# Autodesk Inventor assembly: ロボット回転
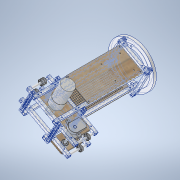
[picture p0: Inventor's stored thumbnail of the model, 180x180]
Saved by Autodesk Inventor 2020.3 (Build 243373000, 373)
## iProperties
Created: 2020-07-04
Part Number: ロボット回転
Document SubType Name: Assembly
Designer: totot
Mass: 887.957 g
Surface Area: 3001.88 cm^2
Volume: 382.741 cm^3
Density: 2.32 g/cm^3
Author: totot
## Documents named in this file (20)
- D:\mysvn\ロボコン\キャチロボ\キャチロボ設計図\ロボット\ハンド\ロボット回転.iam
- D:\mysvn\ロボコン\キャチロボ\キャチロボ設計図\ロボット\共有パーツ\turntable1.ipt
- D:\mysvn\ロボコン\キャチロボ\キャチロボ設計図\ロボット\共有パーツ\turntable2.ipt
- D:\mysvn\ロボコン\キャチロボ\キャチロボ設計図\ロボット\ハンド\ロボット回転9ｘ9_1.ipt
- D:\mysvn\ロボコン\キャチロボ\キャチロボ設計図\ロボット\ハンド\ロボット回転9x9_2.ipt
- D:\mysvn\ロボコン\キャチロボ\キャチロボ設計図\ロボット\ハンド\ロボット回転9x9_3.ipt
- D:\mysvn\ロボコン\キャチロボ\キャチロボ設計図\ロボット\ハンド\ロボット回転t5.5.ipt
- D:\mysvn\ロボコン\キャチロボ\キャチロボ設計図\ロボット\共有パーツ\RS_540.ipt
- D:\mysvn\ロボコン\キャチロボ\キャチロボ設計図\ロボット\共有パーツ\PS1-20_On.ipt
- D:\mysvn\ロボコン\キャチロボ\キャチロボ設計図\ロボット\ハンド\ロボット回転_ベアリングシャフト縦.ipt
- D:\mysvn\ロボコン\キャチロボ\キャチロボ設計図\ロボット\ハンド\ロボット回転_ベアリングシャフト横.ipt
- D:\mysvn\ロボコン\キャチロボ\キャチロボ設計図\ロボット\ハンド\ロボット回転9x9_4.ipt
- D:\mysvn\ロボコン\キャチロボ\キャチロボ設計図\ロボット\ハンド\ハンド_ベアリング_4-8.ipt
- D:\mysvn\ロボコン\キャチロボ\キャチロボ設計図\ロボット\共有パーツ\ベアリング_6-17.ipt
- D:\mysvn\ロボコン\キャチロボ\キャチロボ設計図\ロボット\共有パーツ\ロボット回転_回路ボード1.ipt
- D:\mysvn\ロボコン\キャチロボ\キャチロボ設計図\ロボット\共有パーツ\ロボット回転_回路ボード1_CPY.ipt
- D:\mysvn\ロボコン\キャチロボ\キャチロボ設計図\ロボット\共有パーツ\AMT102-Vwide.ipt
- D:\mysvn\ロボコン\キャチロボ\キャチロボ設計図\ロボット\上下直動\ロボット回転t5.5_2.ipt
- D:\mysvn\ロボコン\キャチロボ\キャチロボ設計図\ロボット\上下直動\ロボット回転_エンコーダシャフト.ipt
- D:\mysvn\ロボコン\キャチロボ\キャチロボ設計図\ロボット\共有パーツ\F606ZZ\F606ZZ.iam
## Components (44 placed, 19 different names)
1. turntable1:1 — 正接:1, フラッシュ:1
2. turntable2:1 — 正接:1, フラッシュ:1, 挿入:1, 挿入:2, 挿入:3, 挿入:4
3. ロボット回転9ｘ9_1:1 — 挿入:1, 挿入:2, 挿入:5, 挿入:7, 挿入:17
4. ロボット回転9ｘ9_1:2 — 挿入:3, 挿入:4, 挿入:6, 挿入:8, 挿入:20, 挿入:66
5. ロボット回転9ｘ9_1:3 — 挿入:7, 挿入:8
6. ロボット回転9ｘ9_1:4 — 挿入:5, 挿入:6, 挿入:18, 挿入:19
7. ロボット回転_ベアリングシャフト縦:1 — 正接:26, 正接:27
8. ロボット回転9x9_2:1 — 挿入:17, 挿入:18, 挿入:24, 角度:1, 挿入:48, 挿入:51, 挿入:60, 挿入:69, 挿入:70, 挿入:78
9. ロボット回転9x9_2:2 — 挿入:19, 挿入:20, 挿入:23, 挿入:49, 挿入:50, 挿入:54
10. ロボット回転9x9_3:1 — フラッシュ:6, 正接:6, 正接:7, フラッシュ:7, 挿入:48, 挿入:49, 挿入:55, 挿入:61
11. ロボット回転t5.5:1 — 挿入:23, 挿入:24, 挿入:25, 挿入:26, 挿入:52, 挿入:53, 挿入:71, 挿入:72
12. RS_540:1 — 挿入:25, 挿入:26, 正接:2, フラッシュ:2
13. PS1-20_On:1 — 正接:2, フラッシュ:2, メイト:12, フラッシュ:16
14. ロボット回転9x9_2:3 — 挿入:44, 挿入:46, 挿入:57, 挿入:66, 挿入:75
15. ロボット回転9x9_2:4 — 角度:1, 挿入:45, 挿入:47, 挿入:59, 挿入:67, 挿入:68, 挿入:77
16. ロボット回転9x9_3:2 — 挿入:46, 挿入:47, 正接:5, フラッシュ:5, 挿入:56, 挿入:58, 挿入:73
17. ロボット回転9x9_3:3 — 挿入:50, 挿入:51, メイト:14, 挿入:76
18. ロボット回転9x9_3:4 — 挿入:44, 挿入:45, 挿入:74
19. ロボット回転_ベアリングシャフト縦:2 — フラッシュ:6, 正接:6, 正接:23
20. ロボット回転_ベアリングシャフト縦:3 — 正接:5, フラッシュ:5, 正接:22
21. ロボット回転_ベアリングシャフト縦:4 — 正接:7, フラッシュ:7, 正接:24, 正接:28
22. ロボット回転_ベアリングシャフト横:1 — 挿入:52, 正接:21
23. ロボット回転_ベアリングシャフト横:2 — 挿入:53, 正接:20
24. ロボット回転9x9_4:1 — 挿入:54, 挿入:55, 挿入:56, 挿入:57
25. ロボット回転9x9_4:2 — 挿入:58, 挿入:59, 挿入:60, 挿入:61
26. ハンド_ベアリング_4-8:1 — メイト:10, 挿入:64
27. ハンド_ベアリング_4-8:2 — メイト:10, フラッシュ:8, 挿入:64, 正接:20, メイト:12
28. ハンド_ベアリング_4-8:3 — メイト:11, フラッシュ:8, 挿入:65
29. ハンド_ベアリング_4-8:4 — メイト:11, 挿入:65, 正接:21
30. ベアリング_6-17:1 — 正接:22, フラッシュ:12, フラッシュ:15
31. ベアリング_6-17:2 — フラッシュ:9, メイト:13, 正接:27, フラッシュ:15
32. ベアリング_6-17:3 — フラッシュ:14, 正接:24, メイト:14
33. ベアリング_6-17:5 — フラッシュ:14, 正接:26, メイト:13
34. ベアリング_6-17:6 — 正接:23, フラッシュ:12
35. ベアリング_6-17:7 — フラッシュ:9, 正接:28
36. ロボット回転_回路ボード1:1 — 挿入:67, 挿入:68
37. ロボット回転_回路ボード1_CPY:1 — 挿入:69, 挿入:70
38. AMT102-Vwide:1 — 挿入:71, 挿入:72, フラッシュ:17
39. PS1-20_On:2 — フラッシュ:16, 正接:30
40. ロボット回転t5.5_2:1 — 挿入:73, 挿入:74, 正接:31, メイト:15
41. ロボット回転_エンコーダシャフト:1 — フラッシュ:17, 正接:30, 正接:32
42. F606ZZ:1 [sub-assembly] — 正接:31, メイト:15, 正接:32
43. ロボット回転9x9_4:3 — 挿入:75, 挿入:76
44. ロボット回転9x9_4:4 — 挿入:77, 挿入:78
## Relationships (86: Insert 49, Tangent 17, Flush 13, Mate 6, Angle 1)
- 正接:1 [Tangent]: turntable1:1 ↔ turntable2:1
- フラッシュ:1 [Flush]: turntable1:1 ↔ turntable2:1
- 挿入:1 [Insert]: turntable2:1 ↔ ロボット回転9ｘ9_1:1
- 挿入:2 [Insert]: turntable2:1 ↔ ロボット回転9ｘ9_1:1
- 挿入:3 [Insert]: turntable2:1 ↔ ロボット回転9ｘ9_1:2
- 挿入:4 [Insert]: turntable2:1 ↔ ロボット回転9ｘ9_1:2
- 挿入:5 [Insert]: ロボット回転9ｘ9_1:1 ↔ ロボット回転9ｘ9_1:4
- 挿入:6 [Insert]: ロボット回転9ｘ9_1:2 ↔ ロボット回転9ｘ9_1:4
- 挿入:7 [Insert]: ロボット回転9ｘ9_1:1 ↔ ロボット回転9ｘ9_1:3
- 挿入:8 [Insert]: ロボット回転9ｘ9_1:2 ↔ ロボット回転9ｘ9_1:3
- 挿入:17 [Insert]: ロボット回転9ｘ9_1:1 ↔ ロボット回転9x9_2:1
- 挿入:18 [Insert]: ロボット回転9ｘ9_1:4 ↔ ロボット回転9x9_2:1
- 挿入:19 [Insert]: ロボット回転9ｘ9_1:4 ↔ ロボット回転9x9_2:2
- 挿入:20 [Insert]: ロボット回転9ｘ9_1:2 ↔ ロボット回転9x9_2:2
- 挿入:23 [Insert]: ロボット回転9x9_2:2 ↔ ロボット回転t5.5:1
- 挿入:24 [Insert]: ロボット回転9x9_2:1 ↔ ロボット回転t5.5:1
- 挿入:25 [Insert]: ロボット回転t5.5:1 ↔ RS_540:1
- 挿入:26 [Insert]: ロボット回転t5.5:1 ↔ RS_540:1
- 正接:2 [Tangent]: RS_540:1 ↔ PS1-20_On:1
- フラッシュ:2 [Flush] (-7 mm): RS_540:1 ↔ PS1-20_On:1
- 角度:1 [Angle] (-180 deg): ロボット回転9x9_2:1 ↔ ロボット回転9x9_2:4
- [Flush]: ロボット回転_ベアリングシャフト縦:1 ↔ ロボット回転9x9_3:4
- [Tangent]: ロボット回転_ベアリングシャフト縦:1 ↔ ロボット回転9x9_3:4
- 挿入:44 [Insert]: ロボット回転9x9_2:3 ↔ ロボット回転9x9_3:4
- 挿入:45 [Insert]: ロボット回転9x9_2:4 ↔ ロボット回転9x9_3:4
- 挿入:46 [Insert]: ロボット回転9x9_2:3 ↔ ロボット回転9x9_3:2
- 挿入:47 [Insert]: ロボット回転9x9_2:4 ↔ ロボット回転9x9_3:2
- 正接:5 [Tangent]: ロボット回転9x9_3:2 ↔ ロボット回転_ベアリングシャフト縦:3
- フラッシュ:5 [Flush]: ロボット回転9x9_3:2 ↔ ロボット回転_ベアリングシャフト縦:3
- フラッシュ:6 [Flush]: ロボット回転9x9_3:1 ↔ ロボット回転_ベアリングシャフト縦:2
- 正接:6 [Tangent]: ロボット回転9x9_3:1 ↔ ロボット回転_ベアリングシャフト縦:2
- 正接:7 [Tangent]: ロボット回転9x9_3:1 ↔ ロボット回転_ベアリングシャフト縦:4
- フラッシュ:7 [Flush]: ロボット回転9x9_3:1 ↔ ロボット回転_ベアリングシャフト縦:4
- 挿入:48 [Insert]: ロボット回転9x9_2:1 ↔ ロボット回転9x9_3:1
- 挿入:49 [Insert]: ロボット回転9x9_2:2 ↔ ロボット回転9x9_3:1
- 挿入:50 [Insert]: ロボット回転9x9_2:2 ↔ ロボット回転9x9_3:3
- 挿入:51 [Insert]: ロボット回転9x9_2:1 ↔ ロボット回転9x9_3:3
- 挿入:52 [Insert]: ロボット回転t5.5:1 ↔ ロボット回転_ベアリングシャフト横:1
- 挿入:53 [Insert]: ロボット回転t5.5:1 ↔ ロボット回転_ベアリングシャフト横:2
- 挿入:54 [Insert]: ロボット回転9x9_2:2 ↔ ロボット回転9x9_4:1
- 挿入:55 [Insert]: ロボット回転9x9_3:1 ↔ ロボット回転9x9_4:1
- 挿入:56 [Insert]: ロボット回転9x9_3:2 ↔ ロボット回転9x9_4:1
- 挿入:57 [Insert]: ロボット回転9x9_2:3 ↔ ロボット回転9x9_4:1
- 挿入:58 [Insert]: ロボット回転9x9_3:2 ↔ ロボット回転9x9_4:2
- 挿入:59 [Insert]: ロボット回転9x9_2:4 ↔ ロボット回転9x9_4:2
- 挿入:60 [Insert]: ロボット回転9x9_2:1 ↔ ロボット回転9x9_4:2
- 挿入:61 [Insert]: ロボット回転9x9_3:1 ↔ ロボット回転9x9_4:2
- メイト:10 [Mate]: ハンド_ベアリング_4-8:1 ↔ ハンド_ベアリング_4-8:2
- メイト:11 [Mate]: ハンド_ベアリング_4-8:3 ↔ ハンド_ベアリング_4-8:4
- フラッシュ:8 [Flush]: ハンド_ベアリング_4-8:2 ↔ ハンド_ベアリング_4-8:3
- 挿入:64 [Insert]: ハンド_ベアリング_4-8:1 ↔ ハンド_ベアリング_4-8:2
- 挿入:65 [Insert]: ハンド_ベアリング_4-8:3 ↔ ハンド_ベアリング_4-8:4
- 正接:20 [Tangent]: ロボット回転_ベアリングシャフト横:2 ↔ ハンド_ベアリング_4-8:2
- メイト:12 [Mate]: PS1-20_On:1 ↔ ハンド_ベアリング_4-8:2
- 正接:21 [Tangent]: ロボット回転_ベアリングシャフト横:1 ↔ ハンド_ベアリング_4-8:4
- 正接:22 [Tangent]: ロボット回転_ベアリングシャフト縦:3 ↔ ベアリング_6-17:1
- 正接:23 [Tangent]: ロボット回転_ベアリングシャフト縦:2 ↔ ベアリング_6-17:6
- フラッシュ:9 [Flush]: ベアリング_6-17:2 ↔ ベアリング_6-17:7
- フラッシュ:12 [Flush]: ベアリング_6-17:1 ↔ ベアリング_6-17:6
- フラッシュ:14 [Flush]: ベアリング_6-17:3 ↔ ベアリング_6-17:5
- 正接:24 [Tangent]: ロボット回転_ベアリングシャフト縦:4 ↔ ベアリング_6-17:3
- 正接:26 [Tangent]: ロボット回転_ベアリングシャフト縦:1 ↔ ベアリング_6-17:5
- メイト:13 [Mate]: ベアリング_6-17:2 ↔ ベアリング_6-17:5
- 正接:27 [Tangent]: ロボット回転_ベアリングシャフト縦:1 ↔ ベアリング_6-17:2
- メイト:14 [Mate] (10 mm): ロボット回転9x9_3:3 ↔ ベアリング_6-17:3
- 挿入:66 [Insert]: ロボット回転9ｘ9_1:2 ↔ ロボット回転9x9_2:3
- 正接:28 [Tangent]: ロボット回転_ベアリングシャフト縦:4 ↔ ベアリング_6-17:7
- 挿入:67 [Insert]: ロボット回転9x9_2:4 ↔ ロボット回転_回路ボード1:1
- 挿入:68 [Insert]: ロボット回転9x9_2:4 ↔ ロボット回転_回路ボード1:1
- 挿入:69 [Insert]: ロボット回転9x9_2:1 ↔ ロボット回転_回路ボード1_CPY:1
- 挿入:70 [Insert]: ロボット回転9x9_2:1 ↔ ロボット回転_回路ボード1_CPY:1
- フラッシュ:15 [Flush]: ベアリング_6-17:1 ↔ ベアリング_6-17:2
- 挿入:71 [Insert]: ロボット回転t5.5:1 ↔ AMT102-Vwide:1
- 挿入:72 [Insert]: ロボット回転t5.5:1 ↔ AMT102-Vwide:1
- 挿入:73 [Insert]: ロボット回転9x9_3:2 ↔ ロボット回転t5.5_2:1
- 挿入:74 [Insert]: ロボット回転9x9_3:4 ↔ ロボット回転t5.5_2:1
- フラッシュ:16 [Flush]: PS1-20_On:1 ↔ PS1-20_On:2
- フラッシュ:17 [Flush]: AMT102-Vwide:1 ↔ ロボット回転_エンコーダシャフト:1
- 正接:30 [Tangent]: PS1-20_On:2 ↔ ロボット回転_エンコーダシャフト:1
- 正接:31 [Tangent]: ロボット回転t5.5_2:1 ↔ F606ZZ:1
- メイト:15 [Mate]: ロボット回転t5.5_2:1 ↔ F606ZZ:1
- 正接:32 [Tangent]: ロボット回転_エンコーダシャフト:1 ↔ F606ZZ:1
- 挿入:75 [Insert]: ロボット回転9x9_2:3 ↔ ロボット回転9x9_4:3
- 挿入:76 [Insert]: ロボット回転9x9_3:3 ↔ ロボット回転9x9_4:3
- 挿入:77 [Insert]: ロボット回転9x9_2:4 ↔ ロボット回転9x9_4:4
- 挿入:78 [Insert]: ロボット回転9x9_2:1 ↔ ロボット回転9x9_4:4
## Named parameters: d51_d7 = 0 mm, d52_d8 = 0 mm
